# Autodesk Inventor assembly: estanteria
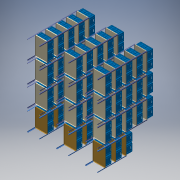
[picture p0: Inventor's stored thumbnail of the model, 180x180]
Saved by Autodesk Inventor 2016 (Build 200138000, 138)
## iProperties
Created: 2015-11-23
Part Number: estanteria
Material: Genérico
Document SubType Name: Assembly
Designer: David
Author: David
## Documents named in this file (4)
- D:\Programas\xampp\htdocs\localUnal\storage\macros\cuarto\Modelado\estanteria.iam
- D:\Programas\xampp\htdocs\localUnal\storage\macros\cuarto\Modelado\estantería\Estante Pequeño\Estante Pequeño.iam
- D:\Programas\xampp\htdocs\localUnal\storage\macros\cuarto\Modelado\estantería\Estantes Grandes\Estante.iam
- D:\Programas\xampp\htdocs\localUnal\storage\macros\cuarto\Modelado\Puente inventor.xlsx
## Components (12 placed, 2 different names)
1. Estante Pequeño:1 [sub-assembly] — Nivelación:1, Nivelación:2, Coincidencia:1
2. Estante Pequeño:2 [sub-assembly]
3. Estante Pequeño:3 [sub-assembly]
4. Estante:1 [sub-assembly] — Nivelación:1, Nivelación:2, Coincidencia:1
5. Estante:2 [sub-assembly]
6. Estante:3 [sub-assembly]
7. Estante:4 [sub-assembly]
8. Estante:5 [sub-assembly]
9. Estante:6 [sub-assembly]
10. Estante:7 [sub-assembly]
11. Estante:8 [sub-assembly]
12. Estante:9 [sub-assembly]
## Component patterns: (3 elements, first: Estante Pequeño:1), (9 elements, first: Estante:1)
## Relationships (3: Flush 2, Mate 1)
- Nivelación:1 [Flush]: Estante Pequeño:1 ↔ Estante:1
- Nivelación:2 [Flush]: Estante Pequeño:1 ↔ Estante:1
- Coincidencia:1 [Mate] (100 mm): Estante Pequeño:1 ↔ Estante:1
## Named parameters: PL_N = 5000 mm, PA_N = 3500 mm, PE_N = 101.6 mm, PL_S = 5000 mm, PA_S = 3500 mm, PE_S = 101.6 mm, DP_S = 3250 mm, AP_S = 2000 mm, PL_EO = 5000 mm, PA_EO = 3500 mm, PE_EO = 101.6 mm, T_L = 5000 mm, T_A = 5000 mm, T_E = 101.6 mm, lon_ve = 512.5 mm, n_a = 3 mm, t_a = 19.05 mm, d_a = 128.125 mm, lon_ho = 749 mm, d_bor = 59.92 mm, lon_gui = 187.25 mm, esp_gui = 461.25 mm, lon_ve2 = 498.475 mm, n_a2 = 3 mm, t_a2 = 124.61875 mm, d_a2 = 124.61875 mm, lon_ho2 = 933.45 mm, d_bor2 = 74.676 mm, lon_gui2 = 233.3625 mm, esp_gui2 = 448.6275 mm, UE_L = 3435 mm, UE_A = 1025 mm, UE_AN = 749 mm, UC_L = 1314.45 mm, UC_A = 996.95 mm, UC_AN = 933.45 mm, A_ET = 35 mm, E_EP = 20 mm, SEP_NS = 0 mm, SEP_EW = 1400 mm, CEP_NS = 1, CEP_EW = 3, DSEG = 0 mm, AEGEP_NS = 0 mm, SEPEG_NS = 100 mm, SEG_NS = 1000 mm, SEG_EW = 1400 mm, CEG_NS = 3, CEG_EW = 3, DNS = 749 mm, DEW = 800 mm
